# Autodesk Inventor assembly: Robot Chassis
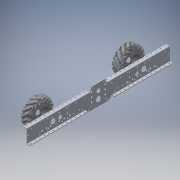
[picture p0: Inventor's stored thumbnail of the model, 180x180]
Saved by Autodesk Inventor 2017 (Build 210142000, 142)
## iProperties
Created: 2017-01-10
Part Number: Robot Chassis
Document SubType Name: Assembly
Designer: Roksbot
Author: Roksbot
## Documents named in this file (4)
- C:\Users\Roksbot\Documents\Inventor\2017 Robot\Robot Chassis.iam
- C:\Users\Roksbot\Documents\Inventor\2017 Robot\am-2952a_AM14U3_Inside_Plate.ipt
- C:\Users\Roksbot\Documents\Inventor\2017 Robot\Left-6-inch-HD-Mecanum-Wheel.ipt
- C:\Users\Roksbot\Documents\Inventor\2017 Robot\Right-6-inch-HD-Mecanum-Wheel.ipt
## Components (3 placed, 3 different names)
1. am-2952a_AM14U3_Inside_Plate:1 — Mate:1, Mate:2, Mate:3, Mate:4, Mate:5
2. Left-6-inch-HD-Mecanum-Wheel:1 — Flush:1, Mate:5
3. Right-6-inch-HD-Mecanum-Wheel:1 — Flush:1, Mate:4
## Relationships (6: Mate 5, Flush 1)
- Mate:1 (-254 mm): am-2952a_AM14U3_Inside_Plate:1
- Mate:2: am-2952a_AM14U3_Inside_Plate:1
- Mate:3: am-2952a_AM14U3_Inside_Plate:1
- Flush:1: Left-6-inch-HD-Mecanum-Wheel:1 ↔ Right-6-inch-HD-Mecanum-Wheel:1
- Mate:4: am-2952a_AM14U3_Inside_Plate:1 ↔ Right-6-inch-HD-Mecanum-Wheel:1
- Mate:5: am-2952a_AM14U3_Inside_Plate:1 ↔ Left-6-inch-HD-Mecanum-Wheel:1
